# Autodesk Inventor assembly: EnsambleFinal
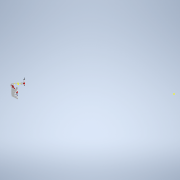
[picture p0: Inventor's stored thumbnail of the model, 180x180]
Saved by Autodesk Inventor 2021 (Build 250183000, 183)
## iProperties
Created: 2022-10-27
Part Number: EnsambleFinal
Document SubType Name: Assembly
Designer: zulet
Author: zulet
## Documents named in this file (20)
- D:\UNAL\2022-2S\Servomecanismos\Proyecto Academico\Servomecanismo2R-main\Servomecanismo2R\INVENTOR\Piezas3D\Piezas3D\EnsambleFinal.iam
- D:\UNAL\2022-2S\Servomecanismos\Proyecto Academico\Motorreductor.ipt
- D:\UNAL\2022-2S\Servomecanismos\Proyecto Academico\Acople4a8.ipt
- D:\UNAL\2022-2S\Servomecanismos\Proyecto Academico\Polea.ipt
- D:\UNAL\2022-2S\Servomecanismos\Proyecto Academico\Eje8.ipt
- C:\Users\zulet\OneDrive\Documents\Inventor\Content Center Files\R2021\en-US\BS 290 SKF(20)\BS 290 SKF - SKF 608-2RZ.ipt
- D:\UNAL\2022-2S\Servomecanismos\Proyecto Academico\Servomecanismo2R-main\Servomecanismo2R\INVENTOR\Piezas3D\Piezas3D\Eslabon1.ipt
- D:\UNAL\2022-2S\Servomecanismos\Proyecto Academico\Servomecanismo2R-main\Servomecanismo2R\INVENTOR\Piezas3D\Piezas3D\Eslabon2.ipt
- D:\UNAL\2022-2S\Servomecanismos\Proyecto Academico\Servomecanismo2R-main\Servomecanismo2R\INVENTOR\Piezas3D\Piezas3D\Eje.ipt
- D:\UNAL\2022-2S\Servomecanismos\Proyecto Academico\Servomecanismo2R-main\Servomecanismo2R\INVENTOR\Piezas3D\Piezas3D\Tensor.ipt
- D:\UNAL\2022-2S\Servomecanismos\Proyecto Academico\AcopleBrida4.ipt
- D:\UNAL\2022-2S\Servomecanismos\Proyecto Academico\AcopleBrida8mm.ipt
- D:\UNAL\2022-2S\Servomecanismos\Proyecto Academico\Servomecanismo2R-main\Servomecanismo2R\INVENTOR\Piezas3D\Piezas3D\Tower Pro MG90S Micro servo\Tower Pro MG90S Micro servo.iam
- D:\UNAL\2022-2S\Servomecanismos\Proyecto Academico\Servomecanismo2R-main\Servomecanismo2R\INVENTOR\Piezas3D\Piezas3D\BaseM1.ipt
- D:\UNAL\2022-2S\Servomecanismos\Proyecto Academico\Servomecanismo2R-main\Servomecanismo2R\INVENTOR\Piezas3D\Piezas3D\SoporteMarcador.ipt
- D:\UNAL\2022-2S\Servomecanismos\Proyecto Academico\Servomecanismo2R-main\Servomecanismo2R\INVENTOR\Piezas3D\Piezas3D\PortaMarcador.ipt
- D:\UNAL\2022-2S\Servomecanismos\Proyecto Academico\Servomecanismo2R-main\Servomecanismo2R\INVENTOR\Piezas3D\Piezas3D\PlacaBase.ipt
- D:\UNAL\2022-2S\Servomecanismos\Proyecto Academico\Servomecanismo2R-main\Servomecanismo2R\INVENTOR\Piezas3D\Piezas3D\marcador.ipt
- C:\Users\zulet\OneDrive\Documents\Inventor\Content Center Files\R2021\en-US\DIN 6912\DIN 6912 - M4 x 12.ipt
- C:\Users\zulet\OneDrive\Documents\Inventor\Content Center Files\R2021\en-US\DIN 7985 (H)\DIN 7985 (H) - M2x6-H.ipt
## Components (23 placed, 19 different names)
1. Motorreductor:1 — Mate:3, Mate:4, Mate:46, Mate:47
2. Acople4a8:1 — Flush:3, Mate:3, Mate:4, Mate:13, Mate:17
3. Eje8:1 — Flush:3, Mate:13, Mate:14, Mate:16
4. BS 290 SKF- with two low-friction seals SKF 608-2RZ:1 — Mate:5, Mate:6, Mate:16, Flush:6
5. Eslabon1:1 — Mate:5, Mate:6, Flush:7, Mate:61, Mate:62, Flush:8, Flush:9, Mate:69
6. Polea:3 — Mate:14, Flush:6, Mate:17
7. AcopleBrida4:1 — Flush:7, Mate:19
8. Motorreductor:2 — Mate:19, Mate:48, Mate:49
9. SoporteMarcador:1
10. PlacaBase:1 — Mate:44, Mate:50, Mate:51, Mate:54, Mate:55, Mate:78
11. DIN 6912 M4 x 12:1 — Mate:44, Mate:52, Mate:55
12. BaseM1:1 — Mate:46, Mate:47, Mate:50, Mate:51, Mate:52
13. BaseM1:2 — Mate:48, Mate:49, Mate:54, Mate:78
14. Eslabon2:1 — Mate:56, Mate:59, Mate:60, Mate:68, Mate:70, Mate:71, Mate:72
15. Tensor:1 — Mate:61, Mate:62, Flush:8, Mate:63, Mate:64
16. Eje:1 — Mate:58, Mate:59, Mate:65, Mate:67, Mate:68
17. Polea:4 — Mate:67, Flush:9
18. BS 290 SKF- with two low-friction seals SKF 608-2RZ:2 — Mate:63, Mate:64, Mate:65
19. AcopleBrida8mm:1 — Mate:56, Mate:58, Mate:60, Mate:69
20. Tower Pro MG90S Micro servo:1 [sub-assembly] — Mate:70, Mate:71, Mate:72, Mate:73, Mate:74
21. PortaMarcador:1 — Mate:73, Mate:75, Mate:76, Mate:77, Flush:10
22. marcador:1 — Mate:77, Flush:10
23. DIN 7985 (H) M2x6-H:1 — Mate:74, Mate:75, Mate:76
## Relationships (46: Mate 40, Flush 6)
- Flush:3: Acople4a8:1 ↔ Eje8:1
- Mate:3: Motorreductor:1 ↔ Acople4a8:1
- Mate:4 (2 mm): Motorreductor:1 ↔ Acople4a8:1
- Mate:5: BS 290 SKF- with two low-friction seals SKF 608-2RZ:1 ↔ Eslabon1:1
- Mate:6: BS 290 SKF- with two low-friction seals SKF 608-2RZ:1 ↔ Eslabon1:1
- Mate:13: Acople4a8:1 ↔ Eje8:1
- Mate:14: Eje8:1 ↔ Polea:3
- Mate:16: Eje8:1 ↔ BS 290 SKF- with two low-friction seals SKF 608-2RZ:1
- Flush:6 (12 mm): BS 290 SKF- with two low-friction seals SKF 608-2RZ:1 ↔ Polea:3
- Mate:17 (9 mm): Acople4a8:1 ↔ Polea:3
- Flush:7: Eslabon1:1 ↔ AcopleBrida4:1
- Mate:19: AcopleBrida4:1 ↔ Motorreductor:2
- Mate:44: PlacaBase:1 ↔ DIN 6912 M4 x 12:1
- Mate:46: Motorreductor:1 ↔ BaseM1:1
- Mate:47: Motorreductor:1 ↔ BaseM1:1
- Mate:48: Motorreductor:2 ↔ BaseM1:2
- Mate:49: Motorreductor:2 ↔ BaseM1:2
- Mate:50: PlacaBase:1 ↔ BaseM1:1
- Mate:51: PlacaBase:1 ↔ BaseM1:1
- Mate:52: DIN 6912 M4 x 12:1 ↔ BaseM1:1
- Mate:54: PlacaBase:1 ↔ BaseM1:2
- Mate:55: PlacaBase:1 ↔ DIN 6912 M4 x 12:1
- Mate:56: Eslabon2:1 ↔ AcopleBrida8mm:1
- Mate:58: Eje:1 ↔ AcopleBrida8mm:1
- Mate:59: Eslabon2:1 ↔ Eje:1
- Mate:60: Eslabon2:1 ↔ AcopleBrida8mm:1
- Mate:61: Eslabon1:1 ↔ Tensor:1
- Mate:62: Eslabon1:1 ↔ Tensor:1
- Flush:8 (10 mm): Eslabon1:1 ↔ Tensor:1
- Mate:63: Tensor:1 ↔ BS 290 SKF- with two low-friction seals SKF 608-2RZ:2
- Mate:64: Tensor:1 ↔ BS 290 SKF- with two low-friction seals SKF 608-2RZ:2
- Mate:65: Eje:1 ↔ BS 290 SKF- with two low-friction seals SKF 608-2RZ:2
- Mate:67: Eje:1 ↔ Polea:4
- Flush:9 (-12 mm): Eslabon1:1 ↔ Polea:4
- Mate:68: Eslabon2:1 ↔ Eje:1
- Mate:69 (5 mm): Eslabon1:1 ↔ AcopleBrida8mm:1
- Mate:70: Eslabon2:1 ↔ Tower Pro MG90S Micro servo:1
- Mate:71: Eslabon2:1 ↔ Tower Pro MG90S Micro servo:1
- Mate:72: Eslabon2:1 ↔ Tower Pro MG90S Micro servo:1
- Mate:73: Tower Pro MG90S Micro servo:1 ↔ PortaMarcador:1
- Mate:74: Tower Pro MG90S Micro servo:1 ↔ DIN 7985 (H) M2x6-H:1
- Mate:75: PortaMarcador:1 ↔ DIN 7985 (H) M2x6-H:1
- Mate:76: PortaMarcador:1 ↔ DIN 7985 (H) M2x6-H:1
- Mate:77: PortaMarcador:1 ↔ marcador:1
- Flush:10 (-20 mm): PortaMarcador:1 ↔ marcador:1
- Mate:78: PlacaBase:1 ↔ BaseM1:2
